# Autodesk Inventor assembly: mock_assembly
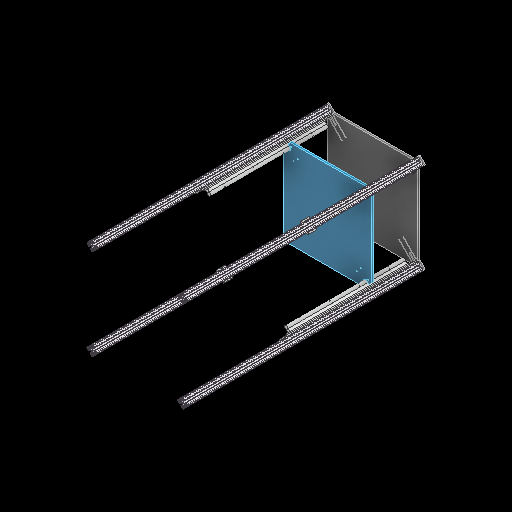
[picture p0: Inventor's stored thumbnail of the model, 512x512]
Saved by Autodesk Inventor 2026.1 (Build 301233000, 233)
## iProperties
Created: 2025-09-21
Part Number: mock_assembly
Document SubType Name: Assembly
Designer: drago
Author: drago
## Documents named in this file (3)
- C:\Users\drago\Desktop\_QIST4500_Multidisciplinary_Team_Project\Proteox MX magnet positioner CAD\mock_assembly.iam
- C:\Users\drago\Desktop\_QIST4500_Multidisciplinary_Team_Project\Proteox MX magnet positioner CAD\gantry_frame\gantry_frame.iam
- C:\Users\drago\Desktop\_QIST4500_Multidisciplinary_Team_Project\Proteox MX magnet positioner CAD\z_plate\z_plate.ipt
## Components (2 placed, 2 different names)
1. gantry_frame:1 [sub-assembly] — Mate:1, Mate:2
2. z_plate:1 — Mate:3, Angle:1
## Relationships (4: Mate 3, Angle 1)
- Mate:1: gantry_frame:1
- Mate:2: gantry_frame:1
- Mate:3: z_plate:1
- Angle:1 (-45 deg): z_plate:1
